# Autodesk Inventor assembly: frame
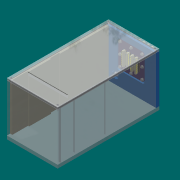
[picture p0: Inventor's stored thumbnail of the model, 180x180]
Saved by Autodesk Inventor 2016 SP1 (Build 200210100, 210)
## iProperties
Created: 2015-10-13
Part Number: frame
Document SubType Name: Assembly
Designer: Sawaiz
Author: Sawaiz
## Documents named in this file (17)
- C:\Users\sawaiz\OneDrive\projects\modularRICH\frame\frame.iam
- C:\Users\sawaiz\OneDrive\projects\modularRICH\frame\leftSide.ipt
- C:\Users\sawaiz\OneDrive\projects\modularRICH\frame\rightSide.ipt
- C:\Users\sawaiz\OneDrive\projects\modularRICH\frame\back.ipt
- C:\Users\sawaiz\OneDrive\projects\modularRICH\frame\bottom.ipt
- C:\Users\sawaiz\OneDrive\projects\modularRICH\frame\front.ipt
- C:\Users\sawaiz\OneDrive\projects\modularRICH\frame\top.ipt
- C:\Users\sawaiz\OneDrive\projects\modularRICH\frame\4-40x0.5in.ipt
- C:\Users\sawaiz\OneDrive\projects\modularRICH\frame\topORing.ipt
- C:\Users\sawaiz\OneDrive\projects\modularRICH\frame\c-51494-2-g.ipt
- C:\Users\sawaiz\OneDrive\projects\modularRICH\frame\backplane\backplane.iam
- C:\Users\sawaiz\OneDrive\projects\modularRICH\frame\backplane\backplaneGasket.ipt
- C:\Users\sawaiz\OneDrive\projects\modularRICH\frame\backplane\2x16IDC.ipt
- C:\Users\sawaiz\OneDrive\projects\modularRICH\frame\frame\AIP\Cable and Harness\frame.Harness1.iam
- C:\Users\sawaiz\OneDrive\projects\modularRICH\frame\no4nut.ipt
- C:\Users\sawaiz\OneDrive\projects\modularRICH\frame\no4washer.ipt
- C:\Users\sawaiz\oneDrive\projects\modularRichFrame\modularRICH.xlsx
## Components (51 placed, 15 different names)
1. leftSide:1 — Flush:1, Flush:2, Flush:9, Flush:10
2. rightSide:1 — Flush:1, Flush:2, Flush:3, Flush:4, Flush:5, Mate:2, Flush:8, Mate:3
3. back:1 — Flush:4, Flush:8, Mate:3, Flush:11, Mate:22, Flush:19, Mate:26, Mate:27, Mate:28, Mate:36, Flush:22, Mate:37, Mate:38, Mate:39, Mate:40, Mate:41, Mate:42, Mate:43
4. bottom:1 — Flush:6, Mate:1, Flush:7
5. front:1 — Flush:3, Flush:5, Flush:6, Mate:1, Flush:7, Mate:2, Flush:9, Mate:11
6. top:1 — Flush:10, Flush:11, Mate:4, Mate:5, Mate:6, Mate:7, Flush:12, Flush:13, Flush:14, Flush:15, Mate:8, Mate:9, Mate:10, Mate:11
7. 4-40x0.5in:1 — Mate:4, Flush:15
8. 4-40x0.5in:2 — Mate:7, Flush:12
9. 4-40x0.5in:3 — Mate:6, Flush:13
10. 4-40x0.5in:4 — Mate:5, Flush:14
11. topORing:1 — Mate:8, Mate:9, Mate:10
12. c-51494-2-g:1 — Mate:22, Flush:19
13. backplane:1 [sub-assembly] — Mate:23, Mate:24, Mate:25, Mate:27, Mate:28, Mate:30, Mate:31, Mate:32, Mate:33, Mate:34, Mate:35, Mate:47
14. backplaneGasket:1 — Mate:23, Mate:24, Mate:25, Mate:26
15. Harness1 [sub-assembly]
16. 4-40x0.5in:5 — Mate:36, Flush:22, Flush:28, Flush:29, Mate:46
17. 4-40x0.5in:6 — Mate:37, Flush:29, Mate:66
18. 4-40x0.5in:7 — Mate:38, Flush:23, Mate:67
19. 4-40x0.5in:8 — Mate:42, Flush:27, Flush:28, Mate:62
20. 4-40x0.5in:9 — Mate:39, Flush:25, Flush:26, Mate:64
21. 4-40x0.5in:10 — Mate:40, Flush:26, Flush:27, Mate:63
22. 4-40x0.5in:11 — Mate:41, Flush:24, Flush:25, Mate:65
23. 4-40x0.5in:12 — Mate:43, Flush:23, Flush:24, Mate:68
24. no4nut:1 — Mate:44, Mate:45, Mate:46, Flush:30
25. no4washer:1 — Mate:44, Mate:45, Mate:47
26. no4nut:2 — Mate:64, Flush:35, Flush:36
27. no4washer:2
28. no4nut:3 — Mate:63, Flush:36, Flush:37
29. no4washer:3
30. no4nut:4 — Mate:65, Flush:34, Flush:35
31. no4washer:4
32. no4nut:5 — Mate:67, Flush:32, Flush:33
33. no4washer:5
34. no4nut:6 — Mate:68, Flush:33, Flush:34
35. no4washer:6
36. no4nut:7 — Mate:66, Flush:31, Flush:32
37. no4washer:7
38. no4nut:8 — Mate:62, Flush:30, Flush:31, Flush:37
39. no4washer:8
40. 2x16IDC:1 — Mate:30, Mate:31, Mate:32
41. 2x16IDC:2
42. 2x16IDC:3
43. 2x16IDC:4 — Flush:20, Flush:21
44. 2x16IDC:5 — Mate:33, Mate:34, Mate:35
45. 2x16IDC:6
46. 2x16IDC:7
47. 2x16IDC:8
48. 2x16IDC:9 — Flush:20, Flush:21
49. 2x16IDC:10
50. 2x16IDC:11
51. 2x16IDC:12
## Component patterns: (4 elements, first: 2x16IDC:1), (4 elements, first: 2x16IDC:5), (4 elements, first: 2x16IDC:9)
## Relationships (91: Mate 57, Flush 34)
- Flush:1: leftSide:1 ↔ rightSide:1
- Flush:2: leftSide:1 ↔ rightSide:1
- Flush:3: rightSide:1 ↔ front:1
- Flush:4: rightSide:1 ↔ back:1
- Flush:5: rightSide:1 ↔ front:1
- Flush:6: bottom:1 ↔ front:1
- Mate:1: bottom:1 ↔ front:1
- Flush:7: bottom:1 ↔ front:1
- Mate:2: rightSide:1 ↔ front:1
- Flush:8: rightSide:1 ↔ back:1
- Mate:3: rightSide:1 ↔ back:1
- Flush:9: leftSide:1 ↔ front:1
- Flush:10: leftSide:1 ↔ top:1
- Flush:11: back:1 ↔ top:1
- Mate:4: top:1 ↔ 4-40x0.5in:1
- Mate:5: top:1 ↔ 4-40x0.5in:4
- Mate:6: top:1 ↔ 4-40x0.5in:3
- Mate:7: top:1 ↔ 4-40x0.5in:2
- Flush:12: top:1 ↔ 4-40x0.5in:2
- Flush:13: top:1 ↔ 4-40x0.5in:3
- Flush:14: top:1 ↔ 4-40x0.5in:4
- Flush:15: top:1 ↔ 4-40x0.5in:1
- Mate:8: top:1 ↔ topORing:1
- Mate:9: top:1 ↔ topORing:1
- Mate:10: top:1 ↔ topORing:1
- Mate:11: front:1 ↔ top:1
- Mate:22: back:1 ↔ c-51494-2-g:1
- Flush:19 (-19.5 mm): back:1 ↔ c-51494-2-g:1
- Mate:23: backplane:1 ↔ backplaneGasket:1
- Mate:24: backplane:1 ↔ backplaneGasket:1
- Mate:25: backplane:1 ↔ backplaneGasket:1
- Mate:26: back:1 ↔ backplaneGasket:1
- Mate:27: back:1 ↔ backplane:1
- Mate:28: back:1 ↔ backplane:1
- Mate:30 (0.05 mm): backplane:1 ↔ 2x16IDC:1
- Mate:31: backplane:1 ↔ 2x16IDC:1
- Mate:32: backplane:1 ↔ 2x16IDC:1
- Mate:33 (0.05 mm): backplane:1 ↔ 2x16IDC:5
- Mate:34 (0.05 mm): backplane:1 ↔ 2x16IDC:5
- Mate:35: backplane:1 ↔ 2x16IDC:5
- Flush:20: 2x16IDC:4 ↔ 2x16IDC:9
- Flush:21: 2x16IDC:4 ↔ 2x16IDC:9
- Mate:36: back:1 ↔ 4-40x0.5in:5
- Flush:22: back:1 ↔ 4-40x0.5in:5
- Mate:37: back:1 ↔ 4-40x0.5in:6
- Mate:38: back:1 ↔ 4-40x0.5in:7
- Mate:39: back:1 ↔ 4-40x0.5in:9
- Mate:40: back:1 ↔ 4-40x0.5in:10
- Mate:41: back:1 ↔ 4-40x0.5in:11
- Mate:42: back:1 ↔ 4-40x0.5in:8
- Mate:43: back:1 ↔ 4-40x0.5in:12
- Flush:23: 4-40x0.5in:7 ↔ 4-40x0.5in:12
- Flush:24: 4-40x0.5in:11 ↔ 4-40x0.5in:12
- Flush:25: 4-40x0.5in:9 ↔ 4-40x0.5in:11
- Flush:26: 4-40x0.5in:9 ↔ 4-40x0.5in:10
- Flush:27: 4-40x0.5in:8 ↔ 4-40x0.5in:10
- Flush:28: 4-40x0.5in:5 ↔ 4-40x0.5in:8
- Flush:29: 4-40x0.5in:5 ↔ 4-40x0.5in:6
- Mate:44: no4nut:1 ↔ no4washer:1
- Mate:45: no4nut:1 ↔ no4washer:1
- Mate:46: 4-40x0.5in:5 ↔ no4nut:1
- Mate:47: backplane:1 ↔ no4washer:1
- [Mate]: no4nut:2 ↔ no4washer:2
- [Mate]: no4nut:2 ↔ no4washer:2
- [Mate]: no4nut:3 ↔ no4washer:3
- [Mate]: no4nut:3 ↔ no4washer:3
- [Mate]: no4nut:4 ↔ no4washer:4
- [Mate]: no4nut:4 ↔ no4washer:4
- [Mate]: no4nut:5 ↔ no4washer:5
- [Mate]: no4nut:5 ↔ no4washer:5
- [Mate]: no4nut:6 ↔ no4washer:6
- [Mate]: no4nut:6 ↔ no4washer:6
- [Mate]: no4nut:7 ↔ no4washer:7
- [Mate]: no4nut:7 ↔ no4washer:7
- [Mate]: no4nut:8 ↔ no4washer:8
- [Mate]: no4nut:8 ↔ no4washer:8
- Mate:62: 4-40x0.5in:8 ↔ no4nut:8
- Mate:63: 4-40x0.5in:10 ↔ no4nut:3
- Mate:64: 4-40x0.5in:9 ↔ no4nut:2
- Mate:65: 4-40x0.5in:11 ↔ no4nut:4
- Mate:66: 4-40x0.5in:6 ↔ no4nut:7
- Mate:67: 4-40x0.5in:7 ↔ no4nut:5
- Mate:68: 4-40x0.5in:12 ↔ no4nut:6
- Flush:30: no4nut:1 ↔ no4nut:8
- Flush:31: no4nut:7 ↔ no4nut:8
- Flush:32: no4nut:5 ↔ no4nut:7
- Flush:33: no4nut:5 ↔ no4nut:6
- Flush:34: no4nut:4 ↔ no4nut:6
- Flush:35: no4nut:2 ↔ no4nut:4
- Flush:36: no4nut:2 ↔ no4nut:3
- Flush:37: no4nut:3 ↔ no4nut:8
## Named parameters: acrylicThickness = 6.35 mm, aerogelThickness = 30 mm, height = 127 mm, width = 127 mm, depth = 273.05 mm, mirrorAngle = 5 deg, detectorWidth = 52 mm, detectorHeight = 52 mm, mirrorThickness = 3.175 mm, fresnelThickness = 0.1 mm, grooveDensity = 100, focalLength = 76.2 mm, ior = 1.49, centerThickness = 1.524 mm, fresnelAngle = 90 deg, fresnelEffectiveDiameter = 152.4 mm, mirrorSuppourtWidth = 38.1 mm, backGrooveBit = 4.8006 mm, sensorHolderWidth = 88.9 mm, sensorHolderSensorWidth = 53.975 mm, sensorHolderSesnorHeight = 53.975 mm, sensorHolderHeight = 88.9 mm, sensorHolderSensorHeight = 53.975 mm, sensorHolderORingGroove = 3.175 mm, sensorHolderORing = 3.175 mm, sensorHolderFlushORingID = 304.8 mm, sensorHolderFlushORing = 3.175 mm, frontBackORingID = 419.1 mm, oRingWidth = 1.5875 mm, sensorHolderORingID = 203.2 mm, topBottomHorizontalMirrorGroove = 12.7 mm, backMirrorGroove = 6.35 mm, mirrorGroove = 19.05 mm, compressionPercent = 40, fresnelChamfer = 6.35 mm, mirrorGrooveFillet = 6.35 mm, mirrorGrooveDrill = 6.35 mm, mirrorGrooveMill = 3.175 mm, fresnelMirrorChamfer = 6.35 mm, detectorOpeningHeight = 76.2 mm, detectorOpeningWidth = 76.2 mm, sensorHolderDepth = 19.05 mm, frameAcrylicThickness = 9.525 mm, internalAcrylicThicnkess = 6.35 mm, aerogelWidth = 110 mm, aerogelHeight = 110 mm, internalAcrylicThickness = 6.35 mm, aerogelClearence = 3.175 mm, backplanePCBHeight = 76.2 mm, backplaneHoleOffsett = 6.35 mm, backplanePCBWidth = 76.2 mm, backplanePostionOffsett = 12.7 mm, d277_d273 = 0 mm, d278_d274 = 0 mm, d279_d273 = 0 mm, d280_d274 = 0 mm, d281_d273 = 0 mm, d282_d274 = 0 mm, d283_d273 = 0 mm, d284_d274 = 0 mm, d285_d273 = 0 mm, d286_d274 = 0 mm, d287_d273 = 0 mm, d288_d274 = 0 mm, d289_d273 = 0 mm, d290_d274 = 0 mm, moduleSlotClearence = 0.79375 mm, testMountWidth = 300 mm, testMountHeight = 300 mm, testMountLength = 500 mm
